# Autodesk Inventor assembly: LiftAssembly_Coupled
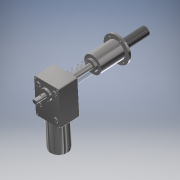
[picture p0: Inventor's stored thumbnail of the model, 180x180]
Saved by Autodesk Inventor 2018 (Build 220112000, 112)
## iProperties
Created: 2018-04-10
Part Number: LiftAssembly_Coupled
Document SubType Name: Assembly
Designer: P136265
Author: P136265
## Documents named in this file (7)
- C:\Users\P136265\Documents\GitHub\mecanum-cad\LiftAssembly_Coupled.iam
- C:\Users\P136265\Documents\GitHub\mecanum-cad\TS-58GZ868D.ipt
- C:\Users\P136265\Documents\GitHub\mecanum-cad\MCLX-12-12-F.ipt
- C:\Users\P136265\Documents\GitHub\mecanum-cad\LeadScrew.ipt
- C:\Users\P136265\Documents\GitHub\mecanum-cad\RNFBL2005A2.5S.ipt
- C:\Users\P136265\Documents\Inventor\Content Center Files\R2018\en-US\ISO 3031(1)\ISO 3031 - 12 x 26 x 2(1).ipt
- C:\Users\P136265\Documents\GitHub\mecanum-cad\ThrustWasher.ipt
## Components (7 placed, 6 different names)
1. TS-58GZ868D:1 — Mate:3, Mate:7, Mate:15
2. MCLX-12-12-F:1 — Mate:3, Mate:4, Mate:7, Mate:9
3. LeadScrew:1 — Mate:4, Mate:9, Mate:11, Mate:17, Mate:28, Mate:29
4. RNFBL2005A2.5S:1 — Mate:11, Mate:17
5. ISO 3031Thrust Needle Roller And Cage Assembly 12 x 26 x 2:2 — Mate:27
6. ThrustWasher:3 — Mate:29
7. ThrustWasher:4 — Mate:27, Mate:28
## Relationships (13: Mate 13)
- Mate:3 (2 mm): TS-58GZ868D:1 ↔ MCLX-12-12-F:1
- Mate:4: MCLX-12-12-F:1 ↔ LeadScrew:1
- Mate:7: TS-58GZ868D:1 ↔ MCLX-12-12-F:1
- Mate:9 (12 mm): MCLX-12-12-F:1 ↔ LeadScrew:1
- Mate:11: LeadScrew:1 ↔ RNFBL2005A2.5S:1
- Mate:15: TS-58GZ868D:1
- Mate:17: LeadScrew:1 ↔ RNFBL2005A2.5S:1
- [Mate] (0.2 mm): ISO 3031Thrust Needle Roller And Cage Assembly 12 x 26 x 2:2 ↔ ThrustWasher:4
- [Mate]: ISO 3031Thrust Needle Roller And Cage Assembly 12 x 26 x 2:2 ↔ ThrustWasher:3
- [Mate] (0.2 mm): ISO 3031Thrust Needle Roller And Cage Assembly 12 x 26 x 2:2 ↔ ThrustWasher:3
- Mate:27: ISO 3031Thrust Needle Roller And Cage Assembly 12 x 26 x 2:2 ↔ ThrustWasher:4
- Mate:28: LeadScrew:1 ↔ ThrustWasher:4
- Mate:29: LeadScrew:1 ↔ ThrustWasher:3
## Named parameters: d34_d31 = 0.2 mm, d35_d32 = 0 mm, d36_d33 = 0.2 mm
